# Autodesk Inventor assembly: endless_assembly
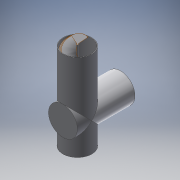
[picture p0: Inventor's stored thumbnail of the model, 180x180]
Saved by Autodesk Inventor 2019 (Build 230136000, 136)
## iProperties
Created: 2019-01-23
Part Number: endless_assembly
Document SubType Name: Assembly
Designer: jmc
Author: jmc
## Documents named in this file (3)
- C:\Users\l0086\Desktop\Models\endless_assembly.iam
- C:\Users\l0086\Desktop\Models\Tests\endless screw\Case.ipt
- C:\Users\l0086\Desktop\Models\Tests\endless screw\Screw.ipt
## Components (2 placed, 2 different names)
1. Case:1 — Rotational:1
2. Screw:1 — Rotational:1
## Relationships (1: RevoluteJoint 1)
- Rotational:1 [RevoluteJoint] (-10 mm): Case:1 ↔ Screw:1
